# Autodesk Inventor assembly: gantry
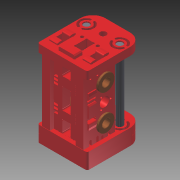
[picture p0: Inventor's stored thumbnail of the model, 180x180]
Saved by Autodesk Inventor 2012 SP1 (Build 160190100, 190)
## iProperties
Created: 2011-11-06
Part Number: gantry
Document SubType Name: Assembly
Designer: Aaron
Author: Aaron
## Documents named in this file (9)
- C:\Users\Aaron\Documents\Projects\MTM-Snap-Metric\gantry.iam
- C:\Users\Aaron\Documents\Projects\MTM-Snap-Metric\gantry7.ipt
- C:\Users\Aaron\Documents\Projects\MTM-Snap-Metric\gantry1.ipt
- C:\Users\Aaron\Documents\Projects\MTM-Snap-Metric\gantry2.ipt
- C:\Users\Aaron\Documents\Projects\MTM-Snap-Metric\gantry3.ipt
- C:\Users\Aaron\Documents\Projects\MTM-Snap-Metric\gantry6.ipt
- C:\Users\Aaron\Documents\Projects\MTM-Snap-Metric\gantry5.ipt
- C:\Users\Aaron\Documents\Projects\InventorParts\Bearing\SHFZ12_25.ipt
- C:\Users\Aaron\Documents\Projects\MTM-Snap-Metric\linear-guide-z.ipt
## Components (12 placed, 8 different names)
1. gantry7:1 — Mate:3, Flush:1, Mate:4, Mate:5, Mate:6, Mate:7, Mate:8, Mate:9
2. gantry1:1 — Mate:3, Flush:1, Mate:4, Mate:5, Mate:6
3. gantry2:1 — Mate:7, Mate:8, Mate:9, Flush:2, Mate:10, Flush:3, Mate:11, Mate:12, Mate:13, Mate:14, Mate:15, Mate:16
4. gantry3:1 — Flush:2, Mate:10, Flush:3, Insert:5, Insert:6
5. gantry6:1 — Mate:11, Mate:12, Mate:13, Insert:3, Insert:4
6. gantry5:1 — Mate:14, Mate:15, Mate:16, Insert:1, Insert:2
7. SHFZ12-25:1 — Insert:1
8. SHFZ12-25:2 — Insert:2
9. SHFZ12-25:3 — Insert:4
10. SHFZ12-25:4 — Insert:3
11. linear-guide-z:1 — Insert:5
12. linear-guide-z:2 — Insert:6
## Relationships (23: Mate 14, Insert 6, Flush 3)
- Mate:3: gantry7:1 ↔ gantry1:1
- Flush:1: gantry7:1 ↔ gantry1:1
- Mate:4: gantry7:1 ↔ gantry1:1
- Mate:5: gantry7:1 ↔ gantry1:1
- Mate:6: gantry7:1 ↔ gantry1:1
- Mate:7: gantry7:1 ↔ gantry2:1
- Mate:8: gantry7:1 ↔ gantry2:1
- Mate:9: gantry7:1 ↔ gantry2:1
- Flush:2: gantry2:1 ↔ gantry3:1
- Mate:10: gantry2:1 ↔ gantry3:1
- Flush:3: gantry2:1 ↔ gantry3:1
- Mate:11: gantry2:1 ↔ gantry6:1
- Mate:12: gantry2:1 ↔ gantry6:1
- Mate:13: gantry2:1 ↔ gantry6:1
- Mate:14: gantry2:1 ↔ gantry5:1
- Mate:15: gantry2:1 ↔ gantry5:1
- Mate:16: gantry2:1 ↔ gantry5:1
- Insert:1: gantry5:1 ↔ SHFZ12-25:1
- Insert:2: gantry5:1 ↔ SHFZ12-25:2
- Insert:3: gantry6:1 ↔ SHFZ12-25:4
- Insert:4: gantry6:1 ↔ SHFZ12-25:3
- Insert:5: gantry3:1 ↔ linear-guide-z:1
- Insert:6: gantry3:1 ↔ linear-guide-z:2
